# Autodesk Inventor assembly: Assembly
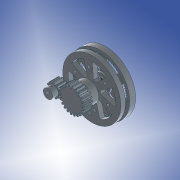
[picture p0: Inventor's stored thumbnail of the model, 180x180]
Saved by Autodesk Inventor 2017 (Build 210142000, 142)
## iProperties
Created: 2017-07-05
Part Number: Assembly
Document SubType Name: Assembly
Designer: zallen
Author: zallen
## Documents named in this file (11)
- C:\Users\zallen\Documents\GitHub\cr-laundry-robot\lib\46_1 Harmonic Drive Gearbox\Assembly.iam
- C:\Users\zallen\Documents\GitHub\cr-laundry-robot\lib\46_1 Harmonic Drive Gearbox\22x8x8mm Bearing.ipt
- C:\Users\zallen\Documents\GitHub\cr-laundry-robot\lib\46_1 Harmonic Drive Gearbox\13x4x5mm Bearing.ipt
- C:\Users\zallen\Documents\GitHub\cr-laundry-robot\lib\46_1 Harmonic Drive Gearbox\Assembly\Design Accelerator\Bolted Connection1.iam
- C:\Users\zallen\Documents\GitHub\cr-laundry-robot\lib\46_1 Harmonic Drive Gearbox\Motor Coupler.ipt
- C:\Users\zallen\Documents\GitHub\cr-laundry-robot\lib\46_1 Harmonic Drive Gearbox\Motor Gear.ipt
- C:\Users\zallen\Documents\GitHub\cr-laundry-robot\lib\46_1 Harmonic Drive Gearbox\Assembly\Design Accelerator\Spur Gears6.iam
- C:\Users\zallen\Documents\GitHub\cr-laundry-robot\lib\46_1 Harmonic Drive Gearbox\BearingCarrier.ipt
- C:\Users\zallen\Documents\GitHub\cr-laundry-robot\lib\46_1 Harmonic Drive Gearbox\Assembly\Design Accelerator\Spur Gears1.iam
- C:\Users\zallen\Documents\Inventor\Content Center Files\R2017\en-US\CNS 3129\CNS 3129 - M 8 x 1.25.ipt
- C:\Users\zallen\Documents\Inventor\Content Center Files\R2017\en-US\ISO 7091\ISO 7091 - ST 8 - 100 HV.ipt
## Components (14 placed, 9 different names)
1. Spur Gears:2 [sub-assembly] — Mate:24, Mate:25, Flush:4, Mate:26, Mate:40
2. 22x8x8mm Bearing:3 — Mate:25, Flush:4, Mate:27, Mate:28, Mate:46
3. Motor Coupler:2 — Mate:29, Mate:30, Mate:32, Rotation:5, Flush:5, Rotation:6, Rotation:7
4. Bolted Connection:2 [sub-assembly] — Mate:27, Mate:28, Mate:29, Mate:30, Mate:33, Mate:39, Rotation:7, Mate:43, Mate:45, Mate:48, Mate:51
5. Motor Gear:2 — Mate:31, Mate:32, Rotation:5, Flush:5
6. BearingCarrier:1 — Mate:33, Mate:35, Mate:36, Mate:37, Mate:38, Rotation:6, Rotation:8, Mate:47, Mate:49
7. 13x4x5mm Bearing:3 — Mate:35, Mate:36
8. 13x4x5mm Bearing:4 — Mate:37, Mate:38
9. Spur Gears:3 [sub-assembly] — Mate:40, Mate:41, Flush:6, Rotation:8
10. 22x8x8mm Bearing:4 — Mate:41, Flush:6, Mate:50, Mate:52
11. CNS 3129 M 8:1 — Mate:43, Mate:53
12. ISO 7091 ST 8 - 100 HV:1 — Mate:45, Mate:46, Mate:47
13. ISO 7091 ST 8 - 100 HV:2 — Mate:51, Mate:52, Mate:53
14. ISO 7091 ST 8 - 100 HV:3 — Mate:48, Mate:49, Mate:50
## Relationships (34: Mate 27, RelateRotation 4, Flush 3)
- Mate:24: Spur Gears:2
- Mate:25: Spur Gears:2 ↔ 22x8x8mm Bearing:3
- Flush:4: Spur Gears:2 ↔ 22x8x8mm Bearing:3
- Mate:26: Spur Gears:2
- Mate:27: 22x8x8mm Bearing:3 ↔ Bolted Connection:2
- Mate:28: 22x8x8mm Bearing:3 ↔ Bolted Connection:2
- Mate:29: Motor Coupler:2 ↔ Bolted Connection:2
- Mate:30: Motor Coupler:2 ↔ Bolted Connection:2
- Mate:31: Motor Gear:2
- Mate:32 (30.5 mm): Motor Coupler:2 ↔ Motor Gear:2
- Rotation:5 [RelateRotation] (0.5 ul): Motor Coupler:2 ↔ Motor Gear:2
- Flush:5: Motor Coupler:2 ↔ Motor Gear:2
- Mate:33: Bolted Connection:2 ↔ BearingCarrier:1
- Mate:35: BearingCarrier:1 ↔ 13x4x5mm Bearing:3
- Mate:36: BearingCarrier:1 ↔ 13x4x5mm Bearing:3
- Mate:37: BearingCarrier:1 ↔ 13x4x5mm Bearing:4
- Mate:38: BearingCarrier:1 ↔ 13x4x5mm Bearing:4
- Mate:39: Bolted Connection:2
- Rotation:6 [RelateRotation] (1 ul): Motor Coupler:2 ↔ BearingCarrier:1
- Rotation:7 [RelateRotation] (1 ul): Motor Coupler:2 ↔ Bolted Connection:2
- Mate:40: Spur Gears:2 ↔ Spur Gears:3
- Mate:41: Spur Gears:3 ↔ 22x8x8mm Bearing:4
- Flush:6: Spur Gears:3 ↔ 22x8x8mm Bearing:4
- Rotation:8 [RelateRotation] (0.0217 ul): BearingCarrier:1 ↔ Spur Gears:3
- Mate:43: Bolted Connection:2 ↔ CNS 3129 M 8:1
- Mate:45: Bolted Connection:2 ↔ ISO 7091 ST 8 - 100 HV:1
- Mate:46: 22x8x8mm Bearing:3 ↔ ISO 7091 ST 8 - 100 HV:1
- Mate:47: BearingCarrier:1 ↔ ISO 7091 ST 8 - 100 HV:1
- Mate:48: Bolted Connection:2 ↔ ISO 7091 ST 8 - 100 HV:3
- Mate:49: BearingCarrier:1 ↔ ISO 7091 ST 8 - 100 HV:3
- Mate:50: 22x8x8mm Bearing:4 ↔ ISO 7091 ST 8 - 100 HV:3
- Mate:51: Bolted Connection:2 ↔ ISO 7091 ST 8 - 100 HV:2
- Mate:52: 22x8x8mm Bearing:4 ↔ ISO 7091 ST 8 - 100 HV:2
- Mate:53: CNS 3129 M 8:1 ↔ ISO 7091 ST 8 - 100 HV:2
